# Autodesk Inventor assembly: ConveyorDriveSide_20Jan
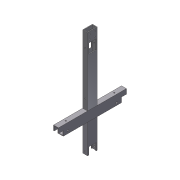
[picture p0: Inventor's stored thumbnail of the model, 180x180]
Saved by Autodesk Inventor 2012 (Build 160160000, 160)
## iProperties
Created: 2012-01-20
Part Number: ConveyorDriveSide_20Jan
Document SubType Name: Assembly
Designer: JesseK
Mass: 743.98 g
Surface Area: 2552.68 cm^2
Volume: 396.136 cm^3
Density: 1.8781 g/cm^3
Author: JesseK
## Documents named in this file (4)
- Z:\UserData\Documents\Inventor\team1885frc\Robot2012\Drawings\ConveyorDriveSide_20Jan.iam
- Z:\UserData\Documents\Inventor\team1885frc\Robot2012\Conveyor2\Frame_MainHorizontalMount.ipt
- Z:\UserData\Documents\Inventor\team1885frc\Robot2012\Conveyor2\Frame_UpperRollerMount.ipt
- Z:\UserData\Documents\Inventor\team1885frc\Robot2012\Conveyor2\Frame_LowerRollerMount.ipt
## Components (3 placed, 3 different names)
1. Frame_MainHorizontalMount:1 — Mate:1, Flush:1, Flush:2, Mate:2, Flush:3
2. Frame_UpperRollerMount:1 — Mate:1, Flush:1, Flush:2, Flush:4
3. Frame_LowerRollerMount:1 — Mate:2, Flush:3, Flush:4
## Relationships (6: Flush 4, Mate 2)
- Mate:1: Frame_MainHorizontalMount:1 ↔ Frame_UpperRollerMount:1
- Flush:1: Frame_MainHorizontalMount:1 ↔ Frame_UpperRollerMount:1
- Flush:2 (152.4 mm): Frame_MainHorizontalMount:1 ↔ Frame_UpperRollerMount:1
- Mate:2: Frame_MainHorizontalMount:1 ↔ Frame_LowerRollerMount:1
- Flush:3: Frame_MainHorizontalMount:1 ↔ Frame_LowerRollerMount:1
- Flush:4: Frame_UpperRollerMount:1 ↔ Frame_LowerRollerMount:1
